# Autodesk Inventor assembly: Robot
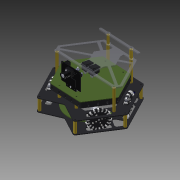
[picture p0: Inventor's stored thumbnail of the model, 180x180]
Saved by Autodesk Inventor 2015 (Build 190159000, 159)
## iProperties
Created: 2016-10-01
Part Number: Robot
Document SubType Name: Assembly
Designer: James Yelland
Author: James Yelland
## Documents named in this file (19)
- C:\Users\James Yelland\git\LJ-STAND\Design\Models\Version 2\Robot.iam
- C:\Users\James Yelland\git\LJ-STAND\Design\Models\Version 2\Bottom Plate.ipt
- C:\Users\James Yelland\git\LJ-STAND\Design\Models\Version 2\Middle Plate.ipt
- C:\Users\James Yelland\git\LJ-STAND\Design\Models\Common\Standoff 30.ipt
- C:\Users\James Yelland\git\LJ-STAND\Design\Models\Version 2\Motor Mount.ipt
- C:\Users\James Yelland\git\LJ-STAND\Design\Models\Common\Motor.ipt
- C:\Users\James Yelland\git\LJ-STAND\Design\Models\Common\Standoff 10.ipt
- C:\Users\James Yelland\git\LJ-STAND\Design\Models\Version 2\PCB.ipt
- C:\Users\James Yelland\git\LJ-STAND\Design\Models\Version 2\TSOP Cover Ring.ipt
- C:\Users\James Yelland\git\LJ-STAND\Design\Models\Version 2\Light Sensor PCB.ipt
- C:\Users\James Yelland\git\LJ-STAND\Design\Models\Version 2\Top Plate.ipt
- C:\Users\James Yelland\git\LJ-STAND\Design\Models\Common\Standoff 20.ipt
- C:\Users\James Yelland\git\LJ-STAND\Design\Models\Version 2\Handle.ipt
- C:\Users\James Yelland\git\LJ-STAND\Design\Models\Common\Standoff 50.ipt
- C:\Users\James Yelland\git\LJ-STAND\Design\Models\Pixy\pixy\Imported Components\Pixy(CMUcam5)\Pixy(CMUcam5).iam
- C:\Users\James Yelland\git\LJ-STAND\Design\Models\Wheel\Wheel.iam
- C:\Users\James Yelland\git\LJ-STAND\Design\Models\Common\Toggle switch.ipt
- C:\Users\James Yelland\git\LJ-STAND\Design\Models\Common\Battery.ipt
- C:\Users\James Yelland\git\LJ-STAND\Design\Models\Common\Pixy angle bracket.ipt
## Components (41 placed, 18 different names)
1. Bottom Plate:1 — Mate:1, Mate:2, Mate:3, Mate:4, Mate:5, Mate:6, Mate:7, Mate:8, Mate:12, Mate:13, Mate:14, Mate:15, Mate:16, Mate:17, Mate:53, Mate:54, Mate:55, Mate:56, Mate:67, Mate:68, Mate:70, Mate:71, Mate:72, Mate:76, Mate:77, Mate:78
2. Middle Plate:1 — Mate:9, Mate:10, Mate:11, Mate:61, Mate:62, Insert:1, Insert:2, Insert:3, Insert:4, Insert:18, Insert:19, Insert:20, Insert:21, Insert:26, Insert:27, Mate:93, Flush:5
3. Standoff 30:1 — Mate:4, Mate:5
4. Standoff 30:2 — Mate:3, Mate:6, Mate:9, Mate:11
5. Standoff 30:3 — Mate:2, Mate:8
6. Standoff 30:4 — Mate:1, Mate:7, Mate:10, Mate:94
7. Motor Mount:1 — Mate:12, Mate:13, Mate:14, Insert:29, Insert:34, Mate:86
8. Motor Mount:2 — Mate:15, Mate:16, Mate:17, Insert:31, Insert:32, Mate:84
9. Standoff 30:5 — Mate:53, Mate:56
10. Standoff 30:6 — Mate:54, Mate:55
11. Standoff 10:1 — Mate:61, Insert:4
12. Standoff 10:2 — Insert:2, Insert:15
13. Standoff 10:3 — Insert:1, Insert:14
14. Standoff 10:4 — Mate:62, Insert:3
15. Light Sensor PCB:1 — Mate:67, Mate:68
16. Top Plate:1 — Insert:10, Insert:11, Insert:22, Insert:23, Mate:87, Mate:88, Mate:89, Mate:90, Mate:91, Mate:92
17. Standoff 20:1 — Insert:10, Insert:12
18. Standoff 20:2 — Insert:11, Insert:13
19. Handle:1 — Insert:12, Insert:13
20. TSOP Cover Ring:1 — Insert:14, Insert:15, Insert:16, Insert:17, Angle:1, Angle:2
21. PCB:1 — Insert:16, Insert:17, Insert:36, Insert:37
22. Standoff 50:1 — Insert:19, Insert:23
23. Standoff 50:2 — Insert:18, Insert:22
24. Standoff 50:3 — Insert:21, Insert:27
25. Standoff 50:4 — Insert:20, Insert:26
26. Pixy(CMUcam5):1 [sub-assembly] — Insert:38, Insert:39
27. Motor Mount:3 — Mate:76, Mate:77, Mate:78, Insert:28, Insert:35, Mate:85
28. Motor Mount:4 — Mate:70, Mate:71, Mate:72, Insert:30, Insert:33, Mate:80
29. Motor:1 — Insert:28, Insert:35, Mate:82
30. Motor:2 — Insert:29, Insert:34, Mate:81
31. Motor:3 — Insert:30, Insert:33, Mate:79
32. Motor:4 — Insert:31, Insert:32, Mate:83
33. Wheel:1 [sub-assembly] — Mate:83, Mate:84
34. Wheel:2 [sub-assembly] — Mate:82, Mate:85
35. Wheel:3 [sub-assembly] — Mate:81, Mate:86
36. Wheel:4 [sub-assembly] — Mate:79, Mate:80
37. Toggle switch:1 — Mate:90, Mate:91, Mate:92
38. Toggle switch:2 — Mate:87, Mate:88, Mate:89
39. Battery:1 — Mate:93, Flush:5, Mate:94
40. Pixy angle bracket:1 — Insert:36, Angle:2, Insert:38
41. Pixy angle bracket:2 — Insert:37, Angle:1, Insert:39
## Relationships (82: Mate 47, Insert 32, Angle 2, Flush 1)
- Mate:1: Bottom Plate:1 ↔ Standoff 30:4
- Mate:2: Bottom Plate:1 ↔ Standoff 30:3
- Mate:3: Bottom Plate:1 ↔ Standoff 30:2
- Mate:4: Bottom Plate:1 ↔ Standoff 30:1
- Mate:5: Bottom Plate:1 ↔ Standoff 30:1
- Mate:6: Bottom Plate:1 ↔ Standoff 30:2
- Mate:7: Bottom Plate:1 ↔ Standoff 30:4
- Mate:8: Bottom Plate:1 ↔ Standoff 30:3
- Mate:9: Middle Plate:1 ↔ Standoff 30:2
- Mate:10: Middle Plate:1 ↔ Standoff 30:4
- Mate:11: Middle Plate:1 ↔ Standoff 30:2
- Mate:12: Bottom Plate:1 ↔ Motor Mount:1
- Mate:13: Bottom Plate:1 ↔ Motor Mount:1
- Mate:14: Bottom Plate:1 ↔ Motor Mount:1
- Mate:15: Bottom Plate:1 ↔ Motor Mount:2
- Mate:16: Bottom Plate:1 ↔ Motor Mount:2
- Mate:17: Bottom Plate:1 ↔ Motor Mount:2
- Mate:53: Bottom Plate:1 ↔ Standoff 30:5
- Mate:54: Bottom Plate:1 ↔ Standoff 30:6
- Mate:55: Bottom Plate:1 ↔ Standoff 30:6
- Mate:56: Bottom Plate:1 ↔ Standoff 30:5
- Mate:61: Middle Plate:1 ↔ Standoff 10:1
- Mate:62: Middle Plate:1 ↔ Standoff 10:4
- Insert:1: Middle Plate:1 ↔ Standoff 10:3
- Insert:2: Middle Plate:1 ↔ Standoff 10:2
- Insert:3: Middle Plate:1 ↔ Standoff 10:4
- Insert:4: Middle Plate:1 ↔ Standoff 10:1
- Mate:67: Bottom Plate:1 ↔ Light Sensor PCB:1
- Mate:68: Bottom Plate:1 ↔ Light Sensor PCB:1
- Insert:10: Top Plate:1 ↔ Standoff 20:1
- Insert:11: Top Plate:1 ↔ Standoff 20:2
- Insert:12: Standoff 20:1 ↔ Handle:1
- Insert:13: Standoff 20:2 ↔ Handle:1
- Insert:14: Standoff 10:3 ↔ TSOP Cover Ring:1
- Insert:15: Standoff 10:2 ↔ TSOP Cover Ring:1
- Insert:16: TSOP Cover Ring:1 ↔ PCB:1
- Insert:17: TSOP Cover Ring:1 ↔ PCB:1
- Insert:18: Middle Plate:1 ↔ Standoff 50:2
- Insert:19: Middle Plate:1 ↔ Standoff 50:1
- Insert:20: Middle Plate:1 ↔ Standoff 50:4
- Insert:21: Middle Plate:1 ↔ Standoff 50:3
- Insert:22: Top Plate:1 ↔ Standoff 50:2
- Insert:23: Top Plate:1 ↔ Standoff 50:1
- Mate:70: Bottom Plate:1 ↔ Motor Mount:4
- Mate:71: Bottom Plate:1 ↔ Motor Mount:4
- Mate:72: Bottom Plate:1 ↔ Motor Mount:4
- Insert:26: Middle Plate:1 ↔ Standoff 50:4
- Insert:27: Middle Plate:1 ↔ Standoff 50:3
- Mate:76: Bottom Plate:1 ↔ Motor Mount:3
- Mate:77: Bottom Plate:1 ↔ Motor Mount:3
- Mate:78: Bottom Plate:1 ↔ Motor Mount:3
- Insert:28: Motor Mount:3 ↔ Motor:1
- Insert:29: Motor Mount:1 ↔ Motor:2
- Insert:30: Motor Mount:4 ↔ Motor:3
- Insert:31: Motor Mount:2 ↔ Motor:4
- Insert:32: Motor Mount:2 ↔ Motor:4
- Insert:33: Motor Mount:4 ↔ Motor:3
- Insert:34: Motor Mount:1 ↔ Motor:2
- Insert:35: Motor Mount:3 ↔ Motor:1
- Mate:79: Motor:3 ↔ Wheel:4
- Mate:80 (5 mm): Motor Mount:4 ↔ Wheel:4
- Mate:81: Motor:2 ↔ Wheel:3
- Mate:82: Motor:1 ↔ Wheel:2
- Mate:83: Motor:4 ↔ Wheel:1
- Mate:84 (5 mm): Motor Mount:2 ↔ Wheel:1
- Mate:85 (5 mm): Motor Mount:3 ↔ Wheel:2
- Mate:86 (5 mm): Motor Mount:1 ↔ Wheel:3
- Mate:87: Top Plate:1 ↔ Toggle switch:2
- Mate:88: Top Plate:1 ↔ Toggle switch:2
- Mate:89: Top Plate:1 ↔ Toggle switch:2
- Mate:90: Top Plate:1 ↔ Toggle switch:1
- Mate:91: Top Plate:1 ↔ Toggle switch:1
- Mate:92: Top Plate:1 ↔ Toggle switch:1
- Mate:93: Middle Plate:1 ↔ Battery:1
- Flush:5 (5 mm): Middle Plate:1 ↔ Battery:1
- Mate:94 (10 mm): Standoff 30:4 ↔ Battery:1
- Insert:36: PCB:1 ↔ Pixy angle bracket:1
- Insert:37: PCB:1 ↔ Pixy angle bracket:2
- Angle:1 (0 deg): TSOP Cover Ring:1 ↔ Pixy angle bracket:2
- Angle:2 (0 deg): TSOP Cover Ring:1 ↔ Pixy angle bracket:1
- Insert:38: Pixy(CMUcam5):1 ↔ Pixy angle bracket:1
- Insert:39: Pixy(CMUcam5):1 ↔ Pixy angle bracket:2
